# Autodesk Inventor assembly: X Carriage Assembly
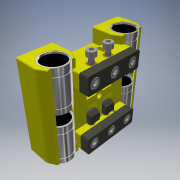
[picture p0: Inventor's stored thumbnail of the model, 180x180]
Saved by Autodesk Inventor 2016 (Build 200138000, 138)
## iProperties
Created: 2017-02-03
Part Number: X Carriage Assembly
Document SubType Name: Assembly
Designer: Scott
Author: Scott
## Documents named in this file (9)
- E:\Scott Projects\3D Printing\CoreXY\X Carriage Assembly.iam
- E:\Scott Projects\3D Printing\CoreXY\X Carriage.ipt
- E:\Scott Projects\3D Printing\CoreXY\M3 Threaded Insert.ipt
- E:\Scott Projects\3D Printing\CoreXY\Belt Tensioner.ipt
- E:\Scott Projects\3D Printing\CoreXY\Belt Clamp.ipt
- C:\Users\Scott\Documents\Inventor\Content Center Files\R2016\en-US\AS 1420\AS 1420 - 1973 - M3 x 10.ipt
- E:\Scott Projects\3D Printing\CoreXY\LM8UU.ipt
- E:\Scott Projects\3D Printing\CoreXY\3x12 Dowel Pin.ipt
- C:\Users\Scott\Documents\Inventor\Content Center Files\R2016\en-US\AS 1420\AS 1420 - 1973 - M3 x 14.ipt
## Components (35 placed, 8 different names)
1. X Carriage:1 — Insert:1, Insert:2, Insert:3, Insert:4, Insert:5, Insert:6, Insert:7, Insert:8, Angle:1, Angle:2, Angle:3, Angle:4, Mate:1, Mate:2, Mate:3, Mate:4, Flush:1, Flush:2, Flush:3, Flush:4, Insert:29, Insert:30, Mate:5, Mate:8, Mate:22, Mate:23, Insert:33, Insert:34, Insert:35, Insert:36
2. M3 Threaded Insert:1 — Insert:4, Mate:10
3. M3 Threaded Insert:2 — Insert:3, Mate:9
4. M3 Threaded Insert:3 — Insert:1, Insert:11
5. M3 Threaded Insert:4 — Insert:2, Insert:12
6. M3 Threaded Insert:5 — Insert:5, Insert:9
7. M3 Threaded Insert:6 — Insert:6, Insert:10
8. M3 Threaded Insert:7 — Insert:7, Mate:6
9. M3 Threaded Insert:8 — Insert:8, Mate:7
10. AS 1420 - Metric M3 x 14:2 — Insert:10, Insert:16
11. AS 1420 - Metric M3 x 14:3 — Insert:9, Insert:15
12. AS 1420 - Metric M3 x 14:4 — Insert:11, Insert:13
13. AS 1420 - Metric M3 x 14:1 — Insert:12, Insert:14
14. Belt Tensioner:1 — Insert:14, Angle:4
15. Belt Tensioner:2 — Insert:13, Angle:2
16. Belt Tensioner:3 — Insert:15, Angle:1
17. Belt Tensioner:4 — Insert:16, Angle:3
18. AS 1420 - Metric M3 x 10:2 — Insert:32
19. LM8UU:1 — Mate:2, Flush:3
20. LM8UU:2 — Mate:1, Flush:1
21. LM8UU:3 — Mate:3, Flush:2
22. LM8UU:4 — Mate:4, Flush:4
23. M3 Threaded Insert:13 — Insert:30
24. M3 Threaded Insert:14 — Insert:29
25. Belt Clamp:1 — Mate:8, Mate:9, Mate:10, Insert:31, Insert:32, Insert:37
26. Belt Clamp:2 — Mate:5, Mate:6, Mate:7, Mate:24, Mate:25, Insert:38
27. AS 1420 - Metric M3 x 10:5 — Insert:31
28. 3x12 Dowel Pin:1 — Insert:35
29. 3x12 Dowel Pin:2 — Insert:36
30. 3x12 Dowel Pin:3 — Insert:34
31. 3x12 Dowel Pin:4 — Insert:33
32. AS 1420 - Metric M3 x 10:6 — Mate:24
33. AS 1420 - Metric M3 x 10:7 — Mate:25
34. AS 1420 - Metric M3 x 10:8 — Insert:37
35. AS 1420 - Metric M3 x 10:9 — Insert:38
## Relationships (48: Insert 26, Mate 14, Angle 4, Flush 4)
- Insert:1: X Carriage:1 ↔ M3 Threaded Insert:3
- Insert:2: X Carriage:1 ↔ M3 Threaded Insert:4
- Insert:3: X Carriage:1 ↔ M3 Threaded Insert:2
- Insert:4: X Carriage:1 ↔ M3 Threaded Insert:1
- Insert:5: X Carriage:1 ↔ M3 Threaded Insert:5
- Insert:6: X Carriage:1 ↔ M3 Threaded Insert:6
- Insert:7: X Carriage:1 ↔ M3 Threaded Insert:7
- Insert:8: X Carriage:1 ↔ M3 Threaded Insert:8
- Insert:9 (4 mm): M3 Threaded Insert:5 ↔ AS 1420 - Metric M3 x 14:3
- Insert:10 (4 mm): M3 Threaded Insert:6 ↔ AS 1420 - Metric M3 x 14:2
- Insert:11 (4 mm): M3 Threaded Insert:3 ↔ AS 1420 - Metric M3 x 14:4
- Insert:12 (4 mm): M3 Threaded Insert:4 ↔ AS 1420 - Metric M3 x 14:1
- Insert:13: AS 1420 - Metric M3 x 14:4 ↔ Belt Tensioner:2
- Insert:14: AS 1420 - Metric M3 x 14:1 ↔ Belt Tensioner:1
- Insert:15: AS 1420 - Metric M3 x 14:3 ↔ Belt Tensioner:3
- Insert:16: AS 1420 - Metric M3 x 14:2 ↔ Belt Tensioner:4
- Angle:1 (0 deg): X Carriage:1 ↔ Belt Tensioner:3
- Angle:2 (0 deg): X Carriage:1 ↔ Belt Tensioner:2
- Angle:3 (0 deg): X Carriage:1 ↔ Belt Tensioner:4
- Angle:4 (0 deg): X Carriage:1 ↔ Belt Tensioner:1
- Mate:1: X Carriage:1 ↔ LM8UU:2
- Mate:2: X Carriage:1 ↔ LM8UU:1
- Mate:3: X Carriage:1 ↔ LM8UU:3
- Mate:4: X Carriage:1 ↔ LM8UU:4
- Flush:1: X Carriage:1 ↔ LM8UU:2
- Flush:2: X Carriage:1 ↔ LM8UU:3
- Flush:3: X Carriage:1 ↔ LM8UU:1
- Flush:4: X Carriage:1 ↔ LM8UU:4
- Insert:29 (1.2 mm): X Carriage:1 ↔ M3 Threaded Insert:14
- Insert:30 (1.2 mm): X Carriage:1 ↔ M3 Threaded Insert:13
- Mate:5: X Carriage:1 ↔ Belt Clamp:2
- Mate:6: M3 Threaded Insert:7 ↔ Belt Clamp:2
- Mate:7: M3 Threaded Insert:8 ↔ Belt Clamp:2
- Mate:8: X Carriage:1 ↔ Belt Clamp:1
- Mate:9: M3 Threaded Insert:2 ↔ Belt Clamp:1
- Mate:10: M3 Threaded Insert:1 ↔ Belt Clamp:1
- Insert:31: Belt Clamp:1 ↔ AS 1420 - Metric M3 x 10:5
- Insert:32: AS 1420 - Metric M3 x 10:2 ↔ Belt Clamp:1
- Mate:22: X Carriage:1
- Mate:23: X Carriage:1
- Insert:33 (-5 mm): X Carriage:1 ↔ 3x12 Dowel Pin:4
- Insert:34 (-5 mm): X Carriage:1 ↔ 3x12 Dowel Pin:3
- Insert:35 (-5 mm): X Carriage:1 ↔ 3x12 Dowel Pin:1
- Insert:36 (-5 mm): X Carriage:1 ↔ 3x12 Dowel Pin:2
- Mate:24: Belt Clamp:2 ↔ AS 1420 - Metric M3 x 10:6
- Mate:25: Belt Clamp:2 ↔ AS 1420 - Metric M3 x 10:7
- Insert:37: Belt Clamp:1 ↔ AS 1420 - Metric M3 x 10:8
- Insert:38: Belt Clamp:2 ↔ AS 1420 - Metric M3 x 10:9
